# Autodesk Inventor assembly: Tattu_Battery_Tray
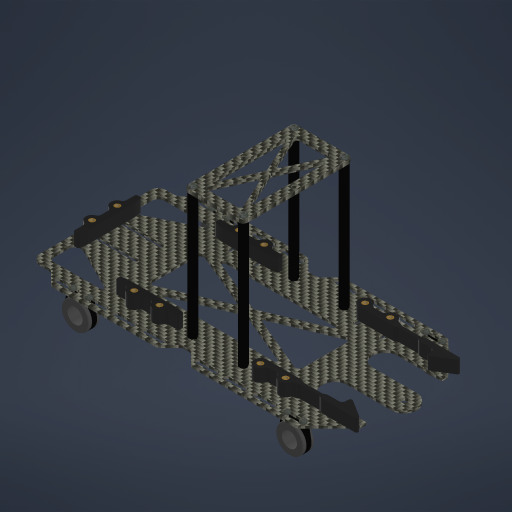
[picture p0: Inventor's stored thumbnail of the model, 512x512]
Saved by Autodesk Inventor 2024 (Build 280153000, 153)
## iProperties
Created: 2023-06-19
Part Number: Tattu_Battery_Tray
Document SubType Name: Assembly
Designer: dzw04
Author: dzw04
## Documents named in this file (9)
- C:\Users\dzw04\Saxion\Mechatronica Lectoraat LMECH LED - Database ARG\Component_Database\SAR\01. CAD\01. 3D_Drawing\02. Sub_Assemblies\Tattu_Battery_Tray.iam
- C:\Users\dzw04\Saxion\Mechatronica Lectoraat LMECH LED - Database ARG\Component_Database\SAR\01. CAD\01. 3D_Drawing\01. Parts\Tattu_Battery_Tray.ipt
- C:\Users\dzw04\Saxion\Mechatronica Lectoraat LMECH LED - Database ARG\Component_Database\SAR\01. CAD\01. 3D_Drawing\02. Sub_Assemblies\Battery_Clip.iam
- C:\Users\dzw04\Saxion\Mechatronica Lectoraat LMECH LED - Database ARG\Component_Database\SAR\01. CAD\01. 3D_Drawing\02. Sub_Assemblies\Battery_Slide.iam
- C:\Users\dzw04\Saxion\Mechatronica Lectoraat LMECH LED - Database ARG\Component_Database\SAR\01. CAD\01. 3D_Drawing\01. Parts\Battery_Standoff.ipt
- C:\Users\dzw04\Saxion\Mechatronica Lectoraat LMECH LED - Database ARG\Component_Database\SAR\01. CAD\01. 3D_Drawing\01. Parts\Tattu_Battery__Top_Tray.ipt
- C:\Users\dzw04\Saxion\Mechatronica Lectoraat LMECH LED - Database ARG\Component_Database\SAR\01. CAD\01. 3D_Drawing\02. Sub_Assemblies\Tarot_12mm_Mount.iam
- C:\Users\dzw04\OneDrive - Saxion\Documenten\Inventor\Content Center Files\R2024\en-US\ISO 7380-1\ISO 7380-1 - M3 x 8.ipt
- C:\Users\dzw04\OneDrive - Saxion\Documenten\Inventor\Content Center Files\R2024\en-US\ISO 7045  Z\ISO 7045 - M2,5 x 5_ - 4.8 - Z - ISO.ipt
## Components (41 placed, 8 different names)
1. Tattu_Battery_Tray:1 — Mate:1, Mate:2, Mate:3, Mate:4, Mate:5, Mate:6, Mate:7, Mate:8, Mate:9, Mate:10, Mate:11, Mate:12, Mate:13, Mate:14, Mate:15, Mate:18, Mate:21, Mate:27, Mate:28, Flush:3, Insert:2, Mate:29, Mate:30, Insert:3, Insert:4, Insert:5, Insert:6, Insert:7, Insert:8, Insert:9, Insert:10, Insert:11, Mate:32, Mate:34
2. Battery_Clip:1 [sub-assembly] — Mate:3, Mate:8, Mate:9
3. Battery_Clip:2 [sub-assembly] — Mate:2, Mate:6, Mate:7
4. Battery_Slide:1 [sub-assembly] — Mate:5, Mate:14, Mate:15
5. Battery_Slide:2 [sub-assembly] — Mate:1, Mate:12, Mate:13
6. Battery_Slide:3 [sub-assembly] — Mate:4, Mate:10, Mate:11
7. Tattu_Battery__Top_Tray:1 — Insert:1
8. ISO 7380-1 M3 x 8:9 — Mate:29, Mate:30
9. ISO 7380-1 M3 x 8:10 — Insert:3
10. ISO 7380-1 M3 x 8:11 — Insert:4
11. ISO 7380-1 M3 x 8:12 — Insert:5
12. ISO 7380-1 M3 x 8:13 — Insert:6
13. ISO 7380-1 M3 x 8:14 — Insert:7
14. ISO 7380-1 M3 x 8:15 — Insert:8
15. ISO 7380-1 M3 x 8:16 — Insert:9
16. ISO 7380-1 M3 x 8:17 — Insert:10
17. ISO 7380-1 M3 x 8:18 — Insert:11
18. ISO 7380-1 M3 x 8:1 — Insert:1
19. ISO 7380-1 M3 x 8:2 — Insert:2
20. Battery_Standoff:1 — Mate:18, Mate:21
21. ISO 7380-1 M3 x 8:3
22. ISO 7380-1 M3 x 8:4
23. Battery_Standoff:2
24. ISO 7380-1 M3 x 8:5
25. ISO 7380-1 M3 x 8:6
26. Battery_Standoff:3
27. ISO 7380-1 M3 x 8:7
28. ISO 7380-1 M3 x 8:8
29. Battery_Standoff:4
30. ISO 7045 Z M2,5 x 5 - 4.8 - Z:2 — Mate:33, Mate:34
31. ISO 7045 Z M2,5 x 5 - 4.8 - Z:1 — Mate:31, Mate:32
32. Tarot_12mm_Mount:1 [sub-assembly] — Mate:27, Mate:28, Flush:3, Mate:31, Mate:33
33. ISO 7045 Z M2,5 x 5 - 4.8 - Z:3
34. ISO 7045 Z M2,5 x 5 - 4.8 - Z:4
35. Tarot_12mm_Mount:2 [sub-assembly]
36. ISO 7045 Z M2,5 x 5 - 4.8 - Z:5
37. ISO 7045 Z M2,5 x 5 - 4.8 - Z:6
38. Tarot_12mm_Mount:3 [sub-assembly]
39. ISO 7045 Z M2,5 x 5 - 4.8 - Z:7
40. ISO 7045 Z M2,5 x 5 - 4.8 - Z:8
41. Tarot_12mm_Mount:4 [sub-assembly]
## Component patterns: (4 elements, first: ISO 7380-1 M3 x 8:1 + ISO 7380-1 M3 x 8:2 + Battery_Standoff:1), (4 elements, first: ISO 7045 Z M2,5 x 5 - 4.8 - Z:2 + ISO 7045 Z M2,5 x 5 - 4.8 - Z:1 + Tarot_12mm_Mount:1)
## Relationships (37: Mate 25, Insert 11, Flush 1)
- Mate:1: Tattu_Battery_Tray:1 ↔ Battery_Slide:2
- Mate:2: Tattu_Battery_Tray:1 ↔ Battery_Clip:2
- Mate:3: Tattu_Battery_Tray:1 ↔ Battery_Clip:1
- Mate:4: Tattu_Battery_Tray:1 ↔ Battery_Slide:3
- Mate:5: Tattu_Battery_Tray:1 ↔ Battery_Slide:1
- Mate:6: Tattu_Battery_Tray:1 ↔ Battery_Clip:2
- Mate:7: Tattu_Battery_Tray:1 ↔ Battery_Clip:2
- Mate:8: Tattu_Battery_Tray:1 ↔ Battery_Clip:1
- Mate:9: Tattu_Battery_Tray:1 ↔ Battery_Clip:1
- Mate:10: Tattu_Battery_Tray:1 ↔ Battery_Slide:3
- Mate:11: Tattu_Battery_Tray:1 ↔ Battery_Slide:3
- Mate:12: Tattu_Battery_Tray:1 ↔ Battery_Slide:2
- Mate:13: Tattu_Battery_Tray:1 ↔ Battery_Slide:2
- Mate:14: Tattu_Battery_Tray:1 ↔ Battery_Slide:1
- Mate:15: Tattu_Battery_Tray:1 ↔ Battery_Slide:1
- Mate:18: Tattu_Battery_Tray:1 ↔ Battery_Standoff:1
- Mate:21: Tattu_Battery_Tray:1 ↔ Battery_Standoff:1
- Mate:27: Tattu_Battery_Tray:1 ↔ Tarot_12mm_Mount:1
- Mate:28: Tattu_Battery_Tray:1 ↔ Tarot_12mm_Mount:1
- Flush:3 (3 mm): Tattu_Battery_Tray:1 ↔ Tarot_12mm_Mount:1
- Insert:1: Tattu_Battery__Top_Tray:1 ↔ ISO 7380-1 M3 x 8:1
- Insert:2: Tattu_Battery_Tray:1 ↔ ISO 7380-1 M3 x 8:2
- Mate:29: Tattu_Battery_Tray:1 ↔ ISO 7380-1 M3 x 8:9
- Mate:30: Tattu_Battery_Tray:1 ↔ ISO 7380-1 M3 x 8:9
- Insert:3: Tattu_Battery_Tray:1 ↔ ISO 7380-1 M3 x 8:10
- Insert:4: Tattu_Battery_Tray:1 ↔ ISO 7380-1 M3 x 8:11
- Insert:5: Tattu_Battery_Tray:1 ↔ ISO 7380-1 M3 x 8:12
- Insert:6: Tattu_Battery_Tray:1 ↔ ISO 7380-1 M3 x 8:13
- Insert:7: Tattu_Battery_Tray:1 ↔ ISO 7380-1 M3 x 8:14
- Insert:8: Tattu_Battery_Tray:1 ↔ ISO 7380-1 M3 x 8:15
- Insert:9: Tattu_Battery_Tray:1 ↔ ISO 7380-1 M3 x 8:16
- Insert:10: Tattu_Battery_Tray:1 ↔ ISO 7380-1 M3 x 8:17
- Insert:11: Tattu_Battery_Tray:1 ↔ ISO 7380-1 M3 x 8:18
- Mate:31: ISO 7045 Z M2,5 x 5 - 4.8 - Z:1 ↔ Tarot_12mm_Mount:1
- Mate:32: Tattu_Battery_Tray:1 ↔ ISO 7045 Z M2,5 x 5 - 4.8 - Z:1
- Mate:33: ISO 7045 Z M2,5 x 5 - 4.8 - Z:2 ↔ Tarot_12mm_Mount:1
- Mate:34: Tattu_Battery_Tray:1 ↔ ISO 7045 Z M2,5 x 5 - 4.8 - Z:2
